# Autodesk Inventor assembly: FrisbeeShooterV03
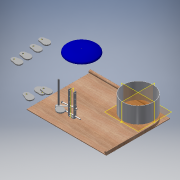
[picture p0: Inventor's stored thumbnail of the model, 180x180]
Saved by Autodesk Inventor 2019.4 (Build 234330000, 330)
## iProperties
Created: 2019-04-25
Part Number: FrisbeeShooterV03
Document SubType Name: Assembly
Designer: steele
Author: steele
## Documents named in this file (9)
- C:\git\CAD-Development\robSteele\2013FrcUltimateAscent\FrisbeeShooterV03.iam
- C:\git\CAD-Development\robSteele\2013FrcUltimateAscent\ShooterBaseV02.ipt
- C:\git\CAD-Development\robSteele\2013FrcUltimateAscent\53214-b_2013.ipt
- C:\git\CAD-Development\robSteele\2013FrcUltimateAscent\FrisbeeHopperV02.ipt
- C:\git\CAD-Development\robSteele\2013FrcUltimateAscent\FrisbeeShooterV02\Design Accelerator\Disc Cam1.iam
- C:\git\CAD-Development\robSteele\2013FrcUltimateAscent\FrisbeeShooterV02\aluminumCamPost.iam
- C:\git\CAD-Development\robSteele\2013FrcUltimateAscent\camPostHolderV03.ipt
- C:\git\CAD-Development\robSteele\2013FrcUltimateAscent\hexShaft.ipt
- C:\git\CAD-Development\robSteele\2013FrcUltimateAscent\FrisbeeShooterV02\Design Accelerator\Disc Cam1.ipt
## Components (21 placed, 7 different names)
1. ShooterBaseV02:1 — Insert:1, Mate:3, Flush:1, Flush:2, Rotational:1, Mate:17, Mate:18
2. 53214-b_2013:1
3. FrisbeeHopperV02:1 — Insert:1
4. Disc Cam:1 [sub-assembly] — Mate:8, Mate:17, Mate:18, Tangent:1
5. camPostHolderV03:1 — Mate:3, Flush:1, Flush:2, Mate:19
6. aluminumCamPost:1 [sub-assembly] — Mate:19, Tangent:1
7. hexShaft:1 — Mate:8, Rotational:1
8. aluminumCamPost:2 [sub-assembly]
9. Disc Cam:2 [sub-assembly]
10. Disc Cam:3
11. Disc Cam:4
12. Disc Cam:5
13. Disc Cam:6
14. Disc Cam:7
15. Disc Cam:8
16. aluminumCamPost:3 [sub-assembly]
17. aluminumCamPost:4 [sub-assembly]
18. aluminumCamPost:5 [sub-assembly]
19. aluminumCamPost:6 [sub-assembly]
20. aluminumCamPost:7 [sub-assembly]
21. aluminumCamPost:8 [sub-assembly]
## Relationships (10: Mate 5, Flush 2, Insert 1, RevoluteJoint 1, Tangent 1)
- Insert:1 (50.8 mm): ShooterBaseV02:1 ↔ FrisbeeHopperV02:1
- Mate:3: ShooterBaseV02:1 ↔ camPostHolderV03:1
- Flush:1 (254 mm): ShooterBaseV02:1 ↔ camPostHolderV03:1
- Flush:2 (152.4 mm): ShooterBaseV02:1 ↔ camPostHolderV03:1
- Mate:8: Disc Cam:1 ↔ hexShaft:1
- Rotational:1 [RevoluteJoint] (-50.8 mm): ShooterBaseV02:1 ↔ hexShaft:1
- Mate:17: ShooterBaseV02:1 ↔ Disc Cam:1
- Mate:18 (14.2875 mm): ShooterBaseV02:1 ↔ Disc Cam:1
- Mate:19: camPostHolderV03:1 ↔ aluminumCamPost:1
- Tangent:1: Disc Cam:1 ↔ aluminumCamPost:1
